# Autodesk Inventor assembly: Mr.Green
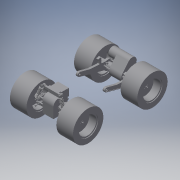
[picture p0: Inventor's stored thumbnail of the model, 180x180]
Saved by Autodesk Inventor 2019 (Build 230136000, 136)
## iProperties
Created: 2019-03-02
Part Number: Mr.Green
Document SubType Name: Assembly
Designer: alarr
Author: alarr
## Documents named in this file (6)
- C:\Users\alarr\OneDrive\Documents\Inventor\Mr.Green\Mr.Green.iam
- C:\Users\alarr\OneDrive\Documents\Inventor\Mr.Green\Back_Wheel_Drive.iam
- C:\Users\alarr\OneDrive\Documents\Inventor\Mr.Green\Wheel.iam
- C:\Users\alarr\OneDrive\Documents\Inventor\Mr.Green\Shock_Arm.ipt
- C:\Users\alarr\OneDrive\Documents\Inventor\Mr.Green\Shock_Arm_MIR.ipt
- C:\Users\alarr\OneDrive\Documents\Inventor\Mr.Green\Front_Wheel_Drive.iam
## Components (8 placed, 5 different names)
1. Back_Wheel_Drive:1 [sub-assembly] — Mate:7, Mate:8, Mate:9, Mate:10, Mate:11, Mate:12, Mate:13, Mate:14, Angle:1, Mate:15, Mate:16, Angle:2
2. Shock_Arm:1 — Mate:7, Mate:8, Mate:9
3. Shock_Arm_MIR:1 — Mate:10, Mate:11, Mate:12
4. Wheel:1 [sub-assembly] — Mate:15, Mate:16, Angle:2
5. Wheel:2 [sub-assembly] — Mate:13, Mate:14, Angle:1
6. Front_Wheel_Drive:1 [sub-assembly] — Mate:17, Mate:18, Angle:3, Mate:19, Mate:20, Angle:4
7. Wheel:3 [sub-assembly] — Mate:17, Mate:18, Angle:3
8. Wheel:4 [sub-assembly] — Mate:19, Mate:20, Angle:4
## Relationships (18: Mate 14, Angle 4)
- Mate:7: Back_Wheel_Drive:1 ↔ Shock_Arm:1
- Mate:8: Back_Wheel_Drive:1 ↔ Shock_Arm:1
- Mate:9: Back_Wheel_Drive:1 ↔ Shock_Arm:1
- Mate:10: Back_Wheel_Drive:1 ↔ Shock_Arm_MIR:1
- Mate:11: Back_Wheel_Drive:1 ↔ Shock_Arm_MIR:1
- Mate:12: Back_Wheel_Drive:1 ↔ Shock_Arm_MIR:1
- Mate:13: Back_Wheel_Drive:1 ↔ Wheel:2
- Mate:14: Back_Wheel_Drive:1 ↔ Wheel:2
- Angle:1 (0 deg): Back_Wheel_Drive:1 ↔ Wheel:2
- Mate:15: Back_Wheel_Drive:1 ↔ Wheel:1
- Mate:16: Back_Wheel_Drive:1 ↔ Wheel:1
- Angle:2 (0 deg): Back_Wheel_Drive:1 ↔ Wheel:1
- Mate:17: Front_Wheel_Drive:1 ↔ Wheel:3
- Mate:18: Front_Wheel_Drive:1 ↔ Wheel:3
- Angle:3 (0 deg): Front_Wheel_Drive:1 ↔ Wheel:3
- Mate:19: Front_Wheel_Drive:1 ↔ Wheel:4
- Mate:20: Front_Wheel_Drive:1 ↔ Wheel:4
- Angle:4 (0 deg): Front_Wheel_Drive:1 ↔ Wheel:4
